# Autodesk Inventor assembly: NP18-12
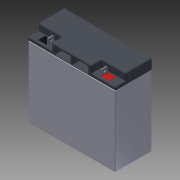
[picture p0: Inventor's stored thumbnail of the model, 180x180]
Saved by Autodesk Inventor 2014 (Build 180170000, 170)
## iProperties
Category: Electrical
Company: Autodesk Inc.
Created: 2011-12-13
Part Number: NP18-12
Document SubType Name: Assembly
Designer: Autodesk
Description: Battery, ,12 volt, 18 AH, Non-spillable
Author: Autodesk Inc.
## Documents named in this file (3)
- C:\Users\steele\Google Drive\FMHS-CAD\CAD Models\Autodesk Parts\2013\Electrical\ELEC_Battery_NP18-12B.iam
- C:\Users\steele\Google Drive\FMHS-CAD\CAD Models\Autodesk Parts\2013\Electrical\Electrical_Yuasa_NP18-12_Top.ipt
- C:\Users\steele\Google Drive\FMHS-CAD\CAD Models\Autodesk Parts\2013\Electrical\Electrical_Yuasa_Np18-12_Middle.ipt
## Components (2 placed, 2 different names)
1. Electrical_Yuasa_NP18-12_Top:1 — Flush:1
2. Electrical_Yuasa_Np18-12_Middle:1 — Flush:1
## Relationships (1: Flush 1)
- Flush:1: Electrical_Yuasa_NP18-12_Top:1 ↔ Electrical_Yuasa_Np18-12_Middle:1
